# Autodesk Inventor assembly: BallShooterV03
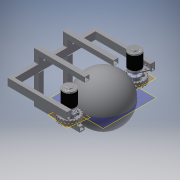
[picture p0: Inventor's stored thumbnail of the model, 180x180]
Saved by Autodesk Inventor 2016 SP1 (Build 200210100, 210)
## iProperties
Created: 2016-01-24
Part Number: BallShooterV03
Document SubType Name: Assembly
Designer: steele
Author: steele
## Documents named in this file (7)
- C:\snobotics\CAD-Development\robSteele\SnoBotics2016\2016-01-28-BallShooter\BallShooterV03.iam
- C:\snobotics\CAD-MfgResources\Andy-Mark\MotorMounts\AM 2488 CIM bracket.ipt
- C:\snobotics\CAD-MfgResources\Andy-Mark\Hubs\am-0320a_8mm_Key_Hub.ipt
- C:\snobotics\CAD-Development\robSteele\SnoBotics2016\DraftOfBoulder.ipt
- C:\snobotics\autodesk\2016\FRC KOP 2016\Motors\MOT_MiniCIMMotor_217-3371.ipt
- C:\snobotics\CAD-Development\robSteele\SnoBotics2016\AM Parts\4 in HiGrip Wheel.iam
- C:\snobotics\CAD-Development\robSteele\SnoBotics2016\2016-01-28-BallShooter\ShooterFrameV03.ipt
## Components (10 placed, 6 different names)
1. ShooterFrameV03:1 — Flush:3, Mate:7, Flush:4, Flush:5, Mate:8, Mate:9, Flush:6, Flush:7
2. AM 2488 CIM bracket:1 — Insert:4, Insert:6, Mate:9, Flush:6, Flush:7
3. MOT_MiniCIMMotor_217-3371:1 — Insert:4
4. am-0320a_8mm_Key_Hub:1 — Insert:6, Insert:10
5. 4 in HiGrip Wheel:1 [sub-assembly] — Insert:10, Mate:10
6. DraftOfBoulder:1 — Flush:3, Mate:8, Mate:10
7. AM 2488 CIM bracket:2 — Mate:7, Flush:4, Flush:5
8. am-0320a_8mm_Key_Hub:2 — Insert:11
9. MOT_MiniCIMMotor_217-3371:2
10. 4 in HiGrip Wheel:2 [sub-assembly] — Insert:11
## Relationships (15: Insert 6, Flush 5, Mate 4)
- Insert:4: AM 2488 CIM bracket:1 ↔ MOT_MiniCIMMotor_217-3371:1
- Insert:6: AM 2488 CIM bracket:1 ↔ am-0320a_8mm_Key_Hub:1
- Flush:3 (254 mm): ShooterFrameV03:1 ↔ DraftOfBoulder:1
- [Insert]: AM 2488 CIM bracket:2 ↔ MOT_MiniCIMMotor_217-3371:2
- [Insert]: AM 2488 CIM bracket:2 ↔ am-0320a_8mm_Key_Hub:2
- Mate:7: ShooterFrameV03:1 ↔ AM 2488 CIM bracket:2
- Flush:4: ShooterFrameV03:1 ↔ AM 2488 CIM bracket:2
- Flush:5: ShooterFrameV03:1 ↔ AM 2488 CIM bracket:2
- Mate:8: ShooterFrameV03:1 ↔ DraftOfBoulder:1
- Mate:9: ShooterFrameV03:1 ↔ AM 2488 CIM bracket:1
- Flush:6: ShooterFrameV03:1 ↔ AM 2488 CIM bracket:1
- Flush:7: ShooterFrameV03:1 ↔ AM 2488 CIM bracket:1
- Insert:10: am-0320a_8mm_Key_Hub:1 ↔ 4 in HiGrip Wheel:1
- Insert:11: am-0320a_8mm_Key_Hub:2 ↔ 4 in HiGrip Wheel:2
- Mate:10: 4 in HiGrip Wheel:1 ↔ DraftOfBoulder:1
## Named parameters: d36_d19 = 0 mm, d38_d26 = 0 mm
